# Autodesk Inventor assembly: Longhouse
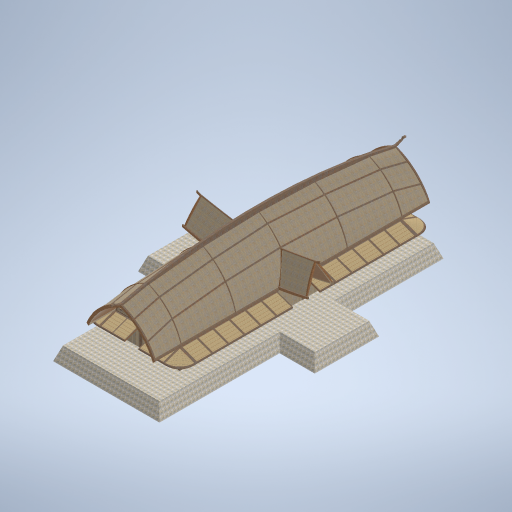
[picture p0: Inventor's stored thumbnail of the model, 512x512]
Saved by Autodesk Inventor 2024.2 (Build 282272000, 272)
## iProperties
Created: 2024-05-22
Part Number: Longhouse
Document SubType Name: Assembly
Designer: LOSTER_1
Author: LOSTER_1
## Documents named in this file (46)
- C:\Users\LOSTER_1\OneDrive\桌面\school\senior\Inventor_Project\Longhouse.iam
- C:\Users\LOSTER_1\OneDrive\桌面\school\senior\Inventor_Project\ROOF\Roof.iam
- C:\Users\LOSTER_1\OneDrive\桌面\school\senior\Inventor_Project\WALL\WallBody.iam
- C:\Users\LOSTER_1\OneDrive\桌面\school\senior\Inventor_Project\ROOF\side_curve_parts\side_curve_beam_01.ipt
- C:\Users\LOSTER_1\OneDrive\桌面\school\senior\Inventor_Project\ROOF\side_curve_parts\side_curve_beam_02.ipt
- C:\Users\LOSTER_1\OneDrive\桌面\school\senior\Inventor_Project\ROOF\side_curve_parts\side_curve_panel_01.ipt
- C:\Users\LOSTER_1\OneDrive\桌面\school\senior\Inventor_Project\ROOF\side_curve_parts\side_curve_beam_03.ipt
- C:\Users\LOSTER_1\OneDrive\桌面\school\senior\Inventor_Project\ROOF\side_curve_parts\side_curve_beam_04.ipt
- C:\Users\LOSTER_1\OneDrive\桌面\school\senior\Inventor_Project\ROOF\side_curve_parts\side_curve_beam_02_MIR.ipt
- C:\Users\LOSTER_1\OneDrive\桌面\school\senior\Inventor_Project\ROOF\side_curve_parts\side_curve_panel_01_MIR.ipt
- C:\Users\LOSTER_1\OneDrive\桌面\school\senior\Inventor_Project\ROOF\side_curve_parts\side_curve_beam_03_MIR.ipt
- C:\Users\LOSTER_1\OneDrive\桌面\school\senior\Inventor_Project\ROOF\side_curve_parts\side_curve_beam_04_MIR.ipt
- C:\Users\LOSTER_1\OneDrive\桌面\school\senior\Inventor_Project\ROOF\side_curve_parts\side_curve_beam_01_MIR.ipt
- C:\Users\LOSTER_1\OneDrive\桌面\school\senior\Inventor_Project\ROOF\side_curve_parts\side_curve_beam_02_MIR1.ipt
- C:\Users\LOSTER_1\OneDrive\桌面\school\senior\Inventor_Project\ROOF\side_curve_parts\side_curve_panel_01_MIR1.ipt
- C:\Users\LOSTER_1\OneDrive\桌面\school\senior\Inventor_Project\ROOF\side_curve_parts\side_curve_beam_03_MIR1.ipt
- C:\Users\LOSTER_1\OneDrive\桌面\school\senior\Inventor_Project\ROOF\side_curve_parts\side_curve_beam_04_MIR1.ipt
- C:\Users\LOSTER_1\OneDrive\桌面\school\senior\Inventor_Project\ROOF\side_curve_parts\side_curve_beam_02_MIR_MIR.ipt
- C:\Users\LOSTER_1\OneDrive\桌面\school\senior\Inventor_Project\ROOF\side_curve_parts\side_curve_panel_01_MIR_MIR.ipt
- C:\Users\LOSTER_1\OneDrive\桌面\school\senior\Inventor_Project\ROOF\side_curve_parts\side_curve_beam_03_MIR_MIR.ipt
- C:\Users\LOSTER_1\OneDrive\桌面\school\senior\Inventor_Project\ROOF\side_curve_parts\side_curve_beam_04_MIR_MIR.ipt
- C:\Users\LOSTER_1\OneDrive\桌面\school\senior\Inventor_Project\ROOF\side_curve_parts_20deg\side_curve_frame_01.ipt
- C:\Users\LOSTER_1\OneDrive\桌面\school\senior\Inventor_Project\ROOF\side_curve_parts_20deg\side_curve_panel_01.ipt
- C:\Users\LOSTER_1\OneDrive\桌面\school\senior\Inventor_Project\ROOF\side_curve_parts_20deg\side_curve_corner_frame.ipt
- C:\Users\LOSTER_1\OneDrive\桌面\school\senior\Inventor_Project\ROOF\side_curve_parts_20deg\side_curve_corner_panel.ipt
- C:\Users\LOSTER_1\OneDrive\桌面\school\senior\Inventor_Project\ROOF\side_curve_parts_20deg\side_curve_frame_02.ipt
- C:\Users\LOSTER_1\OneDrive\桌面\school\senior\Inventor_Project\ROOF\side_curve_parts_20deg\side_curve_panel_02.ipt
- C:\Users\LOSTER_1\OneDrive\桌面\school\senior\Inventor_Project\ROOF\side_curve_parts_20deg\side_curve_frame_01_MIR.ipt
- C:\Users\LOSTER_1\OneDrive\桌面\school\senior\Inventor_Project\ROOF\side_curve_parts_20deg\side_curve_panel_01_MIR.ipt
- C:\Users\LOSTER_1\OneDrive\桌面\school\senior\Inventor_Project\ROOF\side_curve_parts_20deg\side_curve_corner_frame_MIR.ipt
- C:\Users\LOSTER_1\OneDrive\桌面\school\senior\Inventor_Project\ROOF\side_curve_parts_20deg\side_curve_corner_panel_MIR.ipt
- C:\Users\LOSTER_1\OneDrive\桌面\school\senior\Inventor_Project\ROOF\side_curve_parts_20deg\side_curve_frame_02_MIR.ipt
- C:\Users\LOSTER_1\OneDrive\桌面\school\senior\Inventor_Project\ROOF\side_curve_parts_20deg\side_curve_panel_02_MIR.ipt
- C:\Users\LOSTER_1\OneDrive\桌面\school\senior\Inventor_Project\ROOF\side_curve_parts_20deg\side_curve_frame_01_MIR1.ipt
- C:\Users\LOSTER_1\OneDrive\桌面\school\senior\Inventor_Project\ROOF\side_curve_parts_20deg\side_curve_panel_01_MIR1.ipt
- C:\Users\LOSTER_1\OneDrive\桌面\school\senior\Inventor_Project\ROOF\side_curve_parts_20deg\side_curve_corner_frame_MIR1.ipt
- C:\Users\LOSTER_1\OneDrive\桌面\school\senior\Inventor_Project\ROOF\side_curve_parts_20deg\side_curve_corner_panel_MIR1.ipt
- C:\Users\LOSTER_1\OneDrive\桌面\school\senior\Inventor_Project\ROOF\side_curve_parts_20deg\side_curve_frame_02_MIR1.ipt
- C:\Users\LOSTER_1\OneDrive\桌面\school\senior\Inventor_Project\ROOF\side_curve_parts_20deg\side_curve_panel_02_MIR1.ipt
- C:\Users\LOSTER_1\OneDrive\桌面\school\senior\Inventor_Project\ROOF\side_curve_parts_20deg\side_curve_frame_01_MIR_MIR.ipt
- C:\Users\LOSTER_1\OneDrive\桌面\school\senior\Inventor_Project\ROOF\side_curve_parts_20deg\side_curve_panel_01_MIR_MIR.ipt
- C:\Users\LOSTER_1\OneDrive\桌面\school\senior\Inventor_Project\ROOF\side_curve_parts_20deg\side_curve_corner_frame_MIR_MIR.ipt
- C:\Users\LOSTER_1\OneDrive\桌面\school\senior\Inventor_Project\ROOF\side_curve_parts_20deg\side_curve_corner_panel_MIR_MIR.ipt
- C:\Users\LOSTER_1\OneDrive\桌面\school\senior\Inventor_Project\ROOF\side_curve_parts_20deg\side_curve_frame_02_MIR_MIR.ipt
- C:\Users\LOSTER_1\OneDrive\桌面\school\senior\Inventor_Project\ROOF\side_curve_parts_20deg\side_curve_panel_02_MIR_MIR.ipt
- C:\Users\LOSTER_1\OneDrive\桌面\school\senior\Inventor_Project\FLOOR\main_floor.ipt
## Components (89 placed, 41 different names)
1. Roof:1 [sub-assembly] — Mate:1, Flush:2, Mate:125, Mate:126
2. WallBody:1 [sub-assembly] — Mate:1, Flush:1, Mate:130, Mate:131, Mate:132, Mate:133, Mate:134, Mate:135, Mate:136, Mate:137, Mate:138, Mate:139, Mate:140, Mate:141, Mate:154, Mate:157, Mate:158, Mate:159, Mate:218
3. side_curve_beam_01:1 — Mate:125, Mate:128
4. side_curve_beam_02:1 — Mate:126, Mate:127
5. side_curve_panel_01:1 — Mate:127
6. side_curve_beam_03:1
7. side_curve_beam_04:1 — Mate:128
8. side_curve_beam_02_MIR:1
9. side_curve_panel_01_MIR:1
10. side_curve_beam_03_MIR:1
11. side_curve_beam_04_MIR:1
12. side_curve_beam_01_MIR:1 — Mate:129
13. side_curve_beam_02_MIR1:1
14. side_curve_panel_01_MIR1:1
15. side_curve_beam_03_MIR1:1
16. side_curve_beam_04_MIR1:1 — Mate:129
17. side_curve_beam_02_MIR_MIR:1
18. side_curve_panel_01_MIR_MIR:1
19. side_curve_beam_03_MIR_MIR:1
20. side_curve_beam_04_MIR_MIR:1
21. side_curve_frame_01:1 — Mate:130, Mate:131, Mate:142, Mate:143, Mate:155
22. side_curve_frame_01:2 — Mate:132, Mate:133, Mate:144, Mate:145
23. side_curve_frame_01:3 — Mate:134, Mate:135, Mate:146, Mate:147
24. side_curve_frame_01:4 — Mate:136, Mate:137, Mate:148, Mate:149
25. side_curve_frame_01:5 — Mate:138, Mate:139, Mate:150, Mate:151
26. side_curve_frame_01:6 — Mate:140, Mate:141, Mate:152, Mate:153
27. side_curve_panel_01:2 — Mate:142, Mate:143
28. side_curve_panel_01:3 — Mate:144, Mate:145
29. side_curve_panel_01:4 — Mate:146, Mate:147
30. side_curve_panel_01:5 — Mate:148, Mate:149
31. side_curve_panel_01:6 — Mate:150, Mate:151
32. side_curve_panel_01:7 — Mate:152, Mate:153
33. side_curve_corner_frame:1 — Mate:154, Mate:155, Mate:156, Mate:161
34. side_curve_corner_panel:1 — Mate:156
35. side_curve_frame_02:1 — Mate:157, Mate:158, Mate:159, Mate:160, Mate:162, Mate:163
36. side_curve_panel_02:1 — Mate:160, Mate:161
37. side_curve_panel_02:2 — Mate:162, Mate:163
38. side_curve_frame_01_MIR:1 — Mate:164, Mate:165, Mate:176
39. side_curve_frame_01_MIR:2 — Mate:166, Mate:167
40. side_curve_frame_01_MIR:3 — Mate:168, Mate:169
41. side_curve_frame_01_MIR:4 — Mate:170, Mate:171
42. side_curve_frame_01_MIR:5 — Mate:172, Mate:173
43. side_curve_frame_01_MIR:6 — Mate:174, Mate:175
44. side_curve_panel_01_MIR:2 — Mate:164, Mate:165
45. side_curve_panel_01_MIR:3 — Mate:166, Mate:167
46. side_curve_panel_01_MIR:4 — Mate:168, Mate:169
47. side_curve_panel_01_MIR:5 — Mate:170, Mate:171
48. side_curve_panel_01_MIR:6 — Mate:172, Mate:173
49. side_curve_panel_01_MIR:7 — Mate:174, Mate:175
50. side_curve_corner_frame_MIR:1 — Mate:176, Mate:177, Mate:178
51. side_curve_corner_panel_MIR:1 — Mate:177
52. side_curve_frame_02_MIR:1 — Mate:179, Mate:180, Mate:181
53. side_curve_panel_02_MIR:1 — Mate:178, Mate:179
54. side_curve_panel_02_MIR:2 — Mate:180, Mate:181
55. side_curve_frame_01_MIR1:1 — Mate:182, Mate:183, Mate:194
56. side_curve_frame_01_MIR1:2 — Mate:184, Mate:185
57. side_curve_frame_01_MIR1:3 — Mate:186, Mate:187
58. side_curve_frame_01_MIR1:4 — Mate:188, Mate:189
59. side_curve_frame_01_MIR1:5 — Mate:190, Mate:191
60. side_curve_frame_01_MIR1:6 — Mate:192, Mate:193
61. side_curve_panel_01_MIR1:2 — Mate:182, Mate:183
62. side_curve_panel_01_MIR1:3 — Mate:184, Mate:185
63. side_curve_panel_01_MIR1:4 — Mate:186, Mate:187
64. side_curve_panel_01_MIR1:5 — Mate:188, Mate:189
65. side_curve_panel_01_MIR1:6 — Mate:190, Mate:191
66. side_curve_panel_01_MIR1:7 — Mate:192, Mate:193
67. side_curve_corner_frame_MIR1:1 — Mate:194, Mate:195, Mate:196
68. side_curve_corner_panel_MIR1:1 — Mate:195
69. side_curve_frame_02_MIR1:1 — Mate:197, Mate:198, Mate:199
70. side_curve_panel_02_MIR1:1 — Mate:196, Mate:197
71. side_curve_panel_02_MIR1:2 — Mate:198, Mate:199
72. side_curve_frame_01_MIR_MIR:1 — Mate:200, Mate:201, Mate:212
73. side_curve_frame_01_MIR_MIR:2 — Mate:202, Mate:203
74. side_curve_frame_01_MIR_MIR:3 — Mate:204, Mate:205
75. side_curve_frame_01_MIR_MIR:4 — Mate:206, Mate:207
76. side_curve_frame_01_MIR_MIR:5 — Mate:208, Mate:209
77. side_curve_frame_01_MIR_MIR:6 — Mate:210, Mate:211
78. side_curve_panel_01_MIR_MIR:2 — Mate:200, Mate:201
79. side_curve_panel_01_MIR_MIR:3 — Mate:202, Mate:203
80. side_curve_panel_01_MIR_MIR:4 — Mate:204, Mate:205
81. side_curve_panel_01_MIR_MIR:5 — Mate:206, Mate:207
82. side_curve_panel_01_MIR_MIR:6 — Mate:208, Mate:209
83. side_curve_panel_01_MIR_MIR:7 — Mate:210, Mate:211
84. side_curve_corner_frame_MIR_MIR:1 — Mate:212, Mate:213, Mate:215
85. side_curve_corner_panel_MIR_MIR:1 — Mate:213
86. side_curve_frame_02_MIR_MIR:1 — Mate:214, Mate:216, Mate:217
87. side_curve_panel_02_MIR_MIR:1 — Mate:214, Mate:215
88. side_curve_panel_02_MIR_MIR:2 — Mate:216, Mate:217
89. main_floor:1 — Mate:218
## Relationships (97: Mate 95, Flush 2)
- Mate:1: Roof:1 ↔ WallBody:1
- Flush:1: WallBody:1
- Flush:2 (-150 mm): Roof:1
- Mate:125: Roof:1 ↔ side_curve_beam_01:1
- Mate:126: Roof:1 ↔ side_curve_beam_02:1
- Mate:127: side_curve_beam_02:1 ↔ side_curve_panel_01:1
- Mate:128: side_curve_beam_01:1 ↔ side_curve_beam_04:1
- Mate:129: side_curve_beam_01_MIR:1 ↔ side_curve_beam_04_MIR1:1
- Mate:130: WallBody:1 ↔ side_curve_frame_01:1
- Mate:131: WallBody:1 ↔ side_curve_frame_01:1
- Mate:132: WallBody:1 ↔ side_curve_frame_01:2
- Mate:133: WallBody:1 ↔ side_curve_frame_01:2
- Mate:134: WallBody:1 ↔ side_curve_frame_01:3
- Mate:135: WallBody:1 ↔ side_curve_frame_01:3
- Mate:136: WallBody:1 ↔ side_curve_frame_01:4
- Mate:137: WallBody:1 ↔ side_curve_frame_01:4
- Mate:138: WallBody:1 ↔ side_curve_frame_01:5
- Mate:139: WallBody:1 ↔ side_curve_frame_01:5
- Mate:140: WallBody:1 ↔ side_curve_frame_01:6
- Mate:141: WallBody:1 ↔ side_curve_frame_01:6
- Mate:142: side_curve_frame_01:1 ↔ side_curve_panel_01:2
- Mate:143: side_curve_frame_01:1 ↔ side_curve_panel_01:2
- Mate:144: side_curve_frame_01:2 ↔ side_curve_panel_01:3
- Mate:145: side_curve_frame_01:2 ↔ side_curve_panel_01:3
- Mate:146: side_curve_frame_01:3 ↔ side_curve_panel_01:4
- Mate:147: side_curve_frame_01:3 ↔ side_curve_panel_01:4
- Mate:148: side_curve_frame_01:4 ↔ side_curve_panel_01:5
- Mate:149: side_curve_frame_01:4 ↔ side_curve_panel_01:5
- Mate:150: side_curve_frame_01:5 ↔ side_curve_panel_01:6
- Mate:151: side_curve_frame_01:5 ↔ side_curve_panel_01:6
- Mate:152: side_curve_frame_01:6 ↔ side_curve_panel_01:7
- Mate:153: side_curve_frame_01:6 ↔ side_curve_panel_01:7
- Mate:154: WallBody:1 ↔ side_curve_corner_frame:1
- Mate:155: side_curve_frame_01:1 ↔ side_curve_corner_frame:1
- Mate:156: side_curve_corner_frame:1 ↔ side_curve_corner_panel:1
- Mate:157: WallBody:1 ↔ side_curve_frame_02:1
- Mate:158: WallBody:1 ↔ side_curve_frame_02:1
- Mate:159: WallBody:1 ↔ side_curve_frame_02:1
- Mate:160: side_curve_frame_02:1 ↔ side_curve_panel_02:1
- Mate:161: side_curve_corner_frame:1 ↔ side_curve_panel_02:1
- Mate:162: side_curve_frame_02:1 ↔ side_curve_panel_02:2
- Mate:163: side_curve_frame_02:1 ↔ side_curve_panel_02:2
- Mate:164: side_curve_frame_01_MIR:1 ↔ side_curve_panel_01_MIR:2
- Mate:165: side_curve_frame_01_MIR:1 ↔ side_curve_panel_01_MIR:2
- Mate:166: side_curve_frame_01_MIR:2 ↔ side_curve_panel_01_MIR:3
- Mate:167: side_curve_frame_01_MIR:2 ↔ side_curve_panel_01_MIR:3
- Mate:168: side_curve_frame_01_MIR:3 ↔ side_curve_panel_01_MIR:4
- Mate:169: side_curve_frame_01_MIR:3 ↔ side_curve_panel_01_MIR:4
- Mate:170: side_curve_frame_01_MIR:4 ↔ side_curve_panel_01_MIR:5
- Mate:171: side_curve_frame_01_MIR:4 ↔ side_curve_panel_01_MIR:5
- Mate:172: side_curve_frame_01_MIR:5 ↔ side_curve_panel_01_MIR:6
- Mate:173: side_curve_frame_01_MIR:5 ↔ side_curve_panel_01_MIR:6
- Mate:174: side_curve_frame_01_MIR:6 ↔ side_curve_panel_01_MIR:7
- Mate:175: side_curve_frame_01_MIR:6 ↔ side_curve_panel_01_MIR:7
- Mate:176: side_curve_frame_01_MIR:1 ↔ side_curve_corner_frame_MIR:1
- Mate:177: side_curve_corner_frame_MIR:1 ↔ side_curve_corner_panel_MIR:1
- Mate:178: side_curve_corner_frame_MIR:1 ↔ side_curve_panel_02_MIR:1
- Mate:179: side_curve_frame_02_MIR:1 ↔ side_curve_panel_02_MIR:1
- Mate:180: side_curve_frame_02_MIR:1 ↔ side_curve_panel_02_MIR:2
- Mate:181: side_curve_frame_02_MIR:1 ↔ side_curve_panel_02_MIR:2
- Mate:182: side_curve_frame_01_MIR1:1 ↔ side_curve_panel_01_MIR1:2
- Mate:183: side_curve_frame_01_MIR1:1 ↔ side_curve_panel_01_MIR1:2
- Mate:184: side_curve_frame_01_MIR1:2 ↔ side_curve_panel_01_MIR1:3
- Mate:185: side_curve_frame_01_MIR1:2 ↔ side_curve_panel_01_MIR1:3
- Mate:186: side_curve_frame_01_MIR1:3 ↔ side_curve_panel_01_MIR1:4
- Mate:187: side_curve_frame_01_MIR1:3 ↔ side_curve_panel_01_MIR1:4
- Mate:188: side_curve_frame_01_MIR1:4 ↔ side_curve_panel_01_MIR1:5
- Mate:189: side_curve_frame_01_MIR1:4 ↔ side_curve_panel_01_MIR1:5
- Mate:190: side_curve_frame_01_MIR1:5 ↔ side_curve_panel_01_MIR1:6
- Mate:191: side_curve_frame_01_MIR1:5 ↔ side_curve_panel_01_MIR1:6
- Mate:192: side_curve_frame_01_MIR1:6 ↔ side_curve_panel_01_MIR1:7
- Mate:193: side_curve_frame_01_MIR1:6 ↔ side_curve_panel_01_MIR1:7
- Mate:194: side_curve_frame_01_MIR1:1 ↔ side_curve_corner_frame_MIR1:1
- Mate:195: side_curve_corner_frame_MIR1:1 ↔ side_curve_corner_panel_MIR1:1
- Mate:196: side_curve_corner_frame_MIR1:1 ↔ side_curve_panel_02_MIR1:1
- Mate:197: side_curve_frame_02_MIR1:1 ↔ side_curve_panel_02_MIR1:1
- Mate:198: side_curve_frame_02_MIR1:1 ↔ side_curve_panel_02_MIR1:2
- Mate:199: side_curve_frame_02_MIR1:1 ↔ side_curve_panel_02_MIR1:2
- Mate:200: side_curve_frame_01_MIR_MIR:1 ↔ side_curve_panel_01_MIR_MIR:2
- Mate:201: side_curve_frame_01_MIR_MIR:1 ↔ side_curve_panel_01_MIR_MIR:2
- Mate:202: side_curve_frame_01_MIR_MIR:2 ↔ side_curve_panel_01_MIR_MIR:3
- Mate:203: side_curve_frame_01_MIR_MIR:2 ↔ side_curve_panel_01_MIR_MIR:3
- Mate:204: side_curve_frame_01_MIR_MIR:3 ↔ side_curve_panel_01_MIR_MIR:4
- Mate:205: side_curve_frame_01_MIR_MIR:3 ↔ side_curve_panel_01_MIR_MIR:4
- Mate:206: side_curve_frame_01_MIR_MIR:4 ↔ side_curve_panel_01_MIR_MIR:5
- Mate:207: side_curve_frame_01_MIR_MIR:4 ↔ side_curve_panel_01_MIR_MIR:5
- Mate:208: side_curve_frame_01_MIR_MIR:5 ↔ side_curve_panel_01_MIR_MIR:6
- Mate:209: side_curve_frame_01_MIR_MIR:5 ↔ side_curve_panel_01_MIR_MIR:6
- Mate:210: side_curve_frame_01_MIR_MIR:6 ↔ side_curve_panel_01_MIR_MIR:7
- Mate:211: side_curve_frame_01_MIR_MIR:6 ↔ side_curve_panel_01_MIR_MIR:7
- Mate:212: side_curve_frame_01_MIR_MIR:1 ↔ side_curve_corner_frame_MIR_MIR:1
- Mate:213: side_curve_corner_frame_MIR_MIR:1 ↔ side_curve_corner_panel_MIR_MIR:1
- Mate:214: side_curve_frame_02_MIR_MIR:1 ↔ side_curve_panel_02_MIR_MIR:1
- Mate:215: side_curve_corner_frame_MIR_MIR:1 ↔ side_curve_panel_02_MIR_MIR:1
- Mate:216: side_curve_frame_02_MIR_MIR:1 ↔ side_curve_panel_02_MIR_MIR:2
- Mate:217: side_curve_frame_02_MIR_MIR:1 ↔ side_curve_panel_02_MIR_MIR:2
- Mate:218: WallBody:1 ↔ main_floor:1
